# Autodesk Inventor assembly: Assembly1
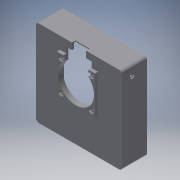
[picture p0: Inventor's stored thumbnail of the model, 180x180]
Saved by Autodesk Inventor 2019 (Build 230136000, 136)
## iProperties
Created: 2020-07-04
Part Number: Assembly1
Document SubType Name: Assembly
Designer: zhang
Author: zhang
## Documents named in this file (3)
- D:\Zhang\Desktop\3D Printing\HyperPixel_case\Assembly1.iam
- D:\Zhang\Desktop\3D Printing\HyperPixel_case\Screen_Top_Open_Back.ipt
- D:\Zhang\Desktop\3D Printing\HyperPixel_case\Cover_w_HQcamera.ipt
## Components (2 placed, 2 different names)
1. Screen_Top_Open_Back:1 — Mate:1, Mate:2, Mate:3
2. Cover_w_HQcamera:1 — Mate:1, Mate:2, Mate:3
## Relationships (3: Mate 3)
- Mate:1: Screen_Top_Open_Back:1 ↔ Cover_w_HQcamera:1
- Mate:2: Screen_Top_Open_Back:1 ↔ Cover_w_HQcamera:1
- Mate:3: Screen_Top_Open_Back:1 ↔ Cover_w_HQcamera:1
